# Autodesk Inventor assembly: Swarmie
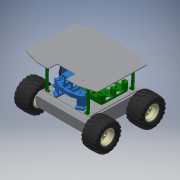
[picture p0: Inventor's stored thumbnail of the model, 180x180]
Saved by Autodesk Inventor 2016 (Build 200138000, 138)
## iProperties
Created: 2015-08-28
Part Number: Swarmie
Document SubType Name: Assembly
Designer: lachesis
Author: lachesis
## Documents named in this file (11)
- C:\Users\lachesis\git\Swarmie-Build\Swarmie Assembly\Assemblies\Swarmie.iam
- C:\Users\lachesis\git\Swarmie-Build\Swarmie Assembly\Assemblies\Chassis.iam
- C:\Users\lachesis\git\Swarmie-Build\Swarmie Assembly\Parts\BatteryBaseSmallLW.ipt
- C:\Users\lachesis\git\Swarmie-Build\Swarmie Assembly\Parts\BatteryBaseLargeLW.ipt
- C:\Users\lachesis\git\Swarmie-Build\Swarmie Assembly\Parts\SingleRegulatorSupport.ipt
- C:\Users\lachesis\git\Swarmie-Build\Swarmie Assembly\Parts\DCMotor.ipt
- C:\Users\lachesis\git\Swarmie-Build\Swarmie Assembly\Parts\MotorHub.ipt
- C:\Users\lachesis\git\Swarmie-Build\Swarmie Assembly\Parts\Tire-Wheel.ipt
- C:\Users\lachesis\git\Swarmie-Build\Swarmie Assembly\Parts\CoverPlate.ipt
- C:\Users\lachesis\git\Swarmie-Build\Swarmie Assembly\Assemblies\TopPlate.iam
- C:\Users\lachesis\git\Swarmie-Build\Swarmie Assembly\Parts\LidSupportLW.ipt
## Components (22 placed, 10 different names)
1. Chassis:1 [sub-assembly] — Rigid:2, Rigid:3, Rotational:1, Rigid:4, Rigid:20, Rigid:18, Rigid:15, Rigid:9
2. BatteryBaseSmallLW:1 — Rigid:2
3. BatteryBaseLargeLW:1 — Rigid:3
4. SingleRegulatorSupport:1 — Rotational:1
5. DCMotor:1 — Rigid:15, Rigid:16
6. DCMotor:2 — Rigid:4, Rigid:17
7. DCMotor:3 — Rigid:18, Rigid:19
8. DCMotor:4 — Rigid:20, Rigid:21
9. MotorHub:1 — Rigid:16, Rigid:5
10. MotorHub:2 — Rigid:19, Rigid:6
11. MotorHub:3 — Rigid:21, Rigid:8
12. MotorHub:4 — Rigid:17, Rigid:7
13. Tire-Wheel:1 — Rigid:5
14. Tire-Wheel:2 — Rigid:6
15. Tire-Wheel:3 — Rigid:7
16. Tire-Wheel:4 — Rigid:8
17. TopPlate:1 [sub-assembly] — Rigid:9, Rigid:10, Rigid:11, Rigid:12, Rigid:13
18. LidSupportLW:1 — Rigid:13
19. LidSupportLW:2 — Rigid:12
20. LidSupportLW:3 — Rigid:11
21. LidSupportLW:4 — Rigid:10
22. CoverPlate:1
## Relationships (20: WeldJoint 19, RevoluteJoint 1)
- Rigid:2 [WeldJoint]: Chassis:1 ↔ BatteryBaseSmallLW:1
- Rigid:3 [WeldJoint]: Chassis:1 ↔ BatteryBaseLargeLW:1
- Rotational:1 [RevoluteJoint]: Chassis:1 ↔ SingleRegulatorSupport:1
- Rigid:4 [WeldJoint]: Chassis:1 ↔ DCMotor:2
- Rigid:20 [WeldJoint]: Chassis:1 ↔ DCMotor:4
- Rigid:18 [WeldJoint]: Chassis:1 ↔ DCMotor:3
- Rigid:15 [WeldJoint]: Chassis:1 ↔ DCMotor:1
- Rigid:16 [WeldJoint] (2.54 mm): DCMotor:1 ↔ MotorHub:1
- Rigid:5 [WeldJoint]: MotorHub:1 ↔ Tire-Wheel:1
- Rigid:19 [WeldJoint] (2.54 mm): DCMotor:3 ↔ MotorHub:2
- Rigid:21 [WeldJoint] (2.54 mm): DCMotor:4 ↔ MotorHub:3
- Rigid:17 [WeldJoint] (-2.54 mm): DCMotor:2 ↔ MotorHub:4
- Rigid:6 [WeldJoint]: MotorHub:2 ↔ Tire-Wheel:2
- Rigid:7 [WeldJoint]: MotorHub:4 ↔ Tire-Wheel:3
- Rigid:8 [WeldJoint]: MotorHub:3 ↔ Tire-Wheel:4
- Rigid:9 [WeldJoint]: Chassis:1 ↔ TopPlate:1
- Rigid:10 [WeldJoint]: TopPlate:1 ↔ LidSupportLW:4
- Rigid:11 [WeldJoint]: TopPlate:1 ↔ LidSupportLW:3
- Rigid:12 [WeldJoint]: TopPlate:1 ↔ LidSupportLW:2
- Rigid:13 [WeldJoint]: TopPlate:1 ↔ LidSupportLW:1
